# Autodesk Inventor assembly: Arm Manipulator
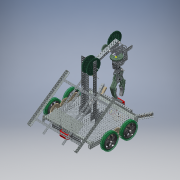
[picture p0: Inventor's stored thumbnail of the model, 180x180]
Saved by Autodesk Inventor 2018 (Build 220112000, 112)
## iProperties
Created: 2018-11-11
Part Number: Arm Manipulator
Document SubType Name: Assembly
Designer: USER
Author: USER
## Documents named in this file (32)
- C:\Users\USER\Desktop\School\Grade 12\Sem 1\Computer Engineering\Competition Robot Inventor\Vex Arm Assembly\Arm Manipulator.iam
- C:\Users\USER\Desktop\School\Grade 12\Sem 1\Computer Engineering\Competition Robot Inventor\Vex Arm Assembly\84 Tooth Gear.ipt
- C:\Users\USER\Desktop\School\Grade 12\Sem 1\Computer Engineering\Competition Robot Inventor\Vex Arm Assembly\Shaft 4 inch.ipt
- C:\Users\USER\Desktop\School\Grade 12\Sem 1\Computer Engineering\Competition Robot Inventor\Vex Arm Assembly\Shaft 3 inch.ipt
- C:\Users\USER\Desktop\School\Grade 12\Sem 1\Computer Engineering\Competition Robot Inventor\Vex Arm Assembly\36 Tooth Gear.ipt
- C:\Users\USER\Desktop\School\Grade 12\Sem 1\Computer Engineering\Competition Robot Inventor\Vex Arm Assembly\Lin Mot-Rack Brk.ipt
- C:\Users\USER\Desktop\School\Grade 12\Sem 1\Computer Engineering\Competition Robot Inventor\Vex Arm Assembly\60 Tooth Gear.ipt
- C:\Users\USER\Desktop\School\Grade 12\Sem 1\Computer Engineering\Competition Robot Inventor\Vex Arm Assembly\Pivot Gusset.ipt
- C:\Users\USER\Desktop\School\Grade 12\Sem 1\Computer Engineering\Competition Robot Inventor\Vex Arm Assembly\Hinge.iam
- C:\Users\USER\Desktop\School\Grade 12\Sem 1\Computer Engineering\Competition Robot Inventor\Vex Arm Assembly\Shaft Collar.iam
- C:\Users\USER\Desktop\School\Grade 12\Sem 1\Computer Engineering\Competition Robot Inventor\Vex Arm Assembly\Screw 8-32  x 0.375 inch long.ipt
- C:\Users\USER\Desktop\School\Grade 12\Sem 1\Computer Engineering\Competition Robot Inventor\Vex Arm Assembly\VEX Claw Finger.iam
- C:\Users\USER\Desktop\School\Grade 12\Sem 1\Computer Engineering\Competition Robot Inventor\Vex Arm Assembly\Gripper_Assembly_SubAssembly.iam
- C:\Users\USER\Desktop\School\Grade 12\Sem 1\Computer Engineering\Competition Robot Inventor\Vex Arm Assembly\VEX-12-TOOTH-GEAR.ipt
- C:\Users\USER\Desktop\School\Grade 12\Sem 1\Computer Engineering\Competition Robot Inventor\Vex Arm Assembly\Vexplorer-CLAW-GEAR-LINKAGE.ipt
- C:\Users\USER\Desktop\School\Grade 12\Sem 1\Computer Engineering\Competition Robot Inventor\Vex Arm Assembly\Vexplorer-CLAW-LINKAGE.ipt
- C:\Users\USER\Desktop\School\Grade 12\Sem 1\Computer Engineering\Competition Robot Inventor\Vex Arm Assembly\SHAFT-2000.ipt
- C:\Users\USER\Desktop\School\Grade 12\Sem 1\Computer Engineering\Competition Robot Inventor\Vex Arm Assembly\Chassis Bumper 25 Hole.ipt
- C:\Users\USER\Desktop\School\Grade 12\Sem 1\Computer Engineering\Competition Robot Inventor\Vex Arm Assembly\Plate 5x25 Hole.ipt
- C:\Users\USER\Downloads\Inventor_2013_VEX_ KOP_-_Metric\Metric\Structure\C-Channel 1x2x1x15 Hole.ipt
- C:\Users\USER\Downloads\Inventor_2013_VEX_ KOP_-_Metric\Metric\Structure\Chassis Rail 25 Hole.ipt
- C:\Users\USER\Downloads\Inventor_2013_VEX_ KOP_-_Metric\Metric\Structure\Bar 1x20.ipt
- C:\Users\USER\Downloads\Inventor_2013_VEX_ KOP_-_Metric\Metric\Motion\Bearing Flat.ipt
- C:\Users\USER\Downloads\Inventor_2013_VEX_ KOP_-_Metric\Metric\Structure\Chassis Rail 16 Hole.ipt
- C:\Users\USER\Downloads\Inventor_2013_VEX_ KOP_-_Metric\Metric\Motion\4 inch Wheel.iam
- C:\Users\USER\Downloads\Inventor_2013_VEX_ KOP_-_Metric\Metric\Motion\19 Tooth Rack Gear.ipt
- C:\Users\USER\Downloads\Inventor_2013_VEX_ KOP_-_Metric\Metric\Structure\Bar 1x25.ipt
- C:\Users\USER\Desktop\School\Grade 12\Sem 1\Computer Engineering\Competition Robot Inventor\Vex Arm Assembly\C-Channel 1x2x1x25 Hole.ipt
- C:\Users\USER\Downloads\Inventor_2013_VEX_ KOP_-_Metric\Metric\Motion\12 Tooth Gear.ipt
- C:\Users\USER\Downloads\Inventor_2013_VEX_ KOP_-_Metric\Metric\Structure\Plate 5x15 Hole.ipt
- C:\Users\USER\Downloads\Inventor_2013_VEX_ KOP_-_Metric\Metric\Sensors\Line Tracker.iam
- C:\Users\USER\Downloads\Inventor_2013_VEX_ KOP_-_Metric\Metric\Sensors\Ultrasonic Range Finder (Sensor).iam
## Components (118 placed, 31 different names)
1. 84 Tooth Gear:1 — Rigid:3, Rigid:11, Rigid:25, Rigid:26, Rotation:4
2. 84 Tooth Gear:2 — Rigid:6
3. 84 Tooth Gear:3 — Rigid:7, Rotation:10
4. Shaft 4 inch:1 — Rigid:3, Rigid:18, Rigid:19, Rotational:42
5. Shaft 4 inch:2 — Rigid:6, Rigid:7, Rigid:21, Rigid:22, Rotational:41, Rigid:42
6. Shaft 3 inch:1 — Rigid:5, Rigid:20, Rigid:31, Rotational:43
7. 36 Tooth Gear:1 — Rigid:5, Flush:1, Rotation:4
8. Lin Mot-Rack Brk:1 — Rotational:4, Rigid:11, Rigid:14
9. Lin Mot-Rack Brk:2 — Rigid:10, Rigid:15, Rigid:29, Rigid:30, Rigid:34
10. 60 Tooth Gear:1 — Rigid:9
11. Shaft 3 inch:2 — Rotational:4, Rigid:9, Rigid:10, Rotational:5, Rigid:23, Rigid:24
12. Pivot Gusset:1 — Rigid:15, Rigid:16
13. Pivot Gusset:2 — Rigid:14
14. Hinge:1 [sub-assembly] — Rigid:17
15. Hinge:2 [sub-assembly] — Rigid:16, Rigid:17
16. Shaft Collar:1 [sub-assembly] — Rigid:19
17. Shaft Collar:2 [sub-assembly] — Rigid:20
18. Shaft Collar:3 [sub-assembly] — Rigid:18
19. Shaft Collar:5 [sub-assembly] — Rigid:21
20. Shaft Collar:6 [sub-assembly] — Rotational:5
21. Shaft Collar:7 [sub-assembly] — Rigid:24
22. Shaft Collar:9 [sub-assembly] — Rigid:23
23. Shaft Collar:10 [sub-assembly] — Rigid:22
24. Hexagon Socket Button Head Cap Screw - Inch 8 - 32 x 3/8:1 — Rigid:26
25. Hexagon Socket Button Head Cap Screw - Inch 8 - 32 x 3/8:3 — Rigid:25
26. Hexagon Socket Button Head Cap Screw - Inch 8 - 32 x 3/8:5 — Rigid:29
27. Hexagon Socket Button Head Cap Screw - Inch 8 - 32 x 3/8:6 — Rigid:30
28. Shaft Collar:11 [sub-assembly] — Rigid:31
29. VEX Claw Finger:1 [sub-assembly] — Rotational:39, Rotational:40
30. VEX Claw Finger:2 [sub-assembly] — Rotational:35, Rotational:36
31. Gripper_Assembly_SubAssembly:1 [sub-assembly] — Rotational:34, Rotational:6, Rotational:7, Rotational:37, Rotational:38, Rigid:34
32. VEX-12-TOOTH-GEAR:1 — Rigid:32, Rotation:2
33. Vexplorer-CLAW-GEAR-LINKAGE:1 — Rotational:37, Rotational:39, Rotation:3
34. Vexplorer-CLAW-LINKAGE:1 — Rotational:38, Rotational:40
35. Vexplorer-CLAW-LINKAGE:2 — Rotational:7, Rotational:36
36. Vexplorer-CLAW-GEAR-LINKAGE:2 — Rotational:6, Rotation:2, Rotational:35, Rotation:3
37. SHAFT-2000:1 — Rigid:32, Rotational:34, Rigid:33
38. Shaft Collar:12 [sub-assembly] — Rigid:33
39. Chassis Bumper 25 Hole:1 — Rigid:41
40. Chassis Bumper 25 Hole:2 — Rotational:41, Rigid:39, Rotational:87
41. Plate 5x25 Hole:1 — Mate:5, Rigid:43, Rigid:50
42. Lin Mot-Rack Brk:3 — Rigid:39, Rigid:43, Rigid:49
43. Lin Mot-Rack Brk:4 — Rigid:41
44. C-Channel 1x2x1x15 Hole:1 — Rotational:42, Rotational:43, Rigid:42
45. Plate 5x25 Hole:2 — Rigid:48, Rigid:53, Rigid:54, Rotational:50, Rotational:86
46. Plate 5x25 Hole:3 — Rigid:49
47. Plate 5x25 Hole:4 — Rigid:51
48. Chassis Rail 25 Hole:1 — Rigid:45, Rigid:46
49. Chassis Rail 25 Hole:2 — Rigid:45, Rigid:48, Rigid:50, Rigid:51, Rigid:52
50. Chassis Rail 25 Hole:3 — Rigid:46, Rigid:47
51. Chassis Rail 25 Hole:4 — Rigid:47, Rigid:89, Rigid:90, Rigid:91
52. Bar 1x20:1 — Rigid:52, Rigid:92
53. Bearing Flat:1 — Rigid:55, Rotational:46
54. Bearing Flat:2 — Rigid:57, Rotational:44
55. Bearing Flat:3 — Rigid:56, Rotational:45
56. Chassis Rail 16 Hole:1 — Rigid:53, Rigid:55, Rigid:56, Rigid:57
57. Chassis Rail 16 Hole:2 — Rigid:54, Rigid:66, Rigid:67, Rigid:68
58. Shaft 4 inch:3 — Rotational:44, Rigid:58, Rigid:61, Rigid:65
59. Shaft 4 inch:4 — Rotational:45, Rigid:60, Rigid:64
60. Shaft 4 inch:5 — Rotational:46, Rigid:59, Rigid:62, Rigid:63
61. 4 inch Wheel:1 [sub-assembly] — Rigid:61
62. Shaft Collar:13 [sub-assembly] — Rigid:58
63. Shaft Collar:14 [sub-assembly] — Rigid:60
64. Shaft Collar:15 [sub-assembly] — Rigid:59
65. 4 inch Wheel:2 [sub-assembly] — Rigid:62
66. 60 Tooth Gear:2 — Rigid:63, Rotation:6
67. 60 Tooth Gear:3 — Rigid:64, Rotation:5, Rotation:6
68. 60 Tooth Gear:4 — Rigid:65, Rotation:5
69. Bearing Flat:4 — Rigid:66, Rotational:47
70. Bearing Flat:5 — Rigid:67, Rotational:48
71. Bearing Flat:6 — Rigid:68, Rotational:49
72. Shaft 4 inch:6 — Rotational:47, Rigid:69, Rigid:72, Rigid:74
73. Shaft 4 inch:7 — Rotational:48, Rigid:70, Rigid:75
74. Shaft 4 inch:8 — Rotational:49, Rigid:71, Rigid:73, Rigid:76
75. Shaft Collar:16 [sub-assembly] — Rigid:69
76. Shaft Collar:17 [sub-assembly] — Rigid:70
77. Shaft Collar:18 [sub-assembly] — Rigid:71
78. 4 inch Wheel:3 [sub-assembly] — Rigid:73
79. 4 inch Wheel:4 [sub-assembly] — Rigid:72
80. 60 Tooth Gear:5 — Rigid:74, Rotation:8
81. 60 Tooth Gear:6 — Rigid:75, Rotation:7, Rotation:8
82. 60 Tooth Gear:7 — Rigid:76, Rotation:7
83. C-Channel 1x2x1x15 Hole:2 — Rigid:77, Rigid:79, Rigid:87
84. C-Channel 1x2x1x15 Hole:3 — Rigid:78, Rigid:80, Rigid:88
85. 60 Tooth Gear:8 — Rigid:77, Rotation:9
86. 60 Tooth Gear:9 — Rigid:78, Rotation:9
87. Bearing Flat:7 — Rigid:79, Rigid:81
88. Bearing Flat:8 — Rigid:80, Rigid:82
89. Shaft 3 inch:3 — Rigid:82, Rigid:84, Rotational:86, Rigid:85
90. Shaft 3 inch:4 — Rigid:81, Rigid:83, Rotational:50, Rigid:86
91. Shaft Collar:19 [sub-assembly] — Rigid:83
92. Shaft Collar:20 [sub-assembly] — Rigid:84
93. Shaft Collar:21 [sub-assembly] — Rigid:85
94. Shaft Collar:22 [sub-assembly] — Rigid:86
95. 19 Tooth Rack Gear:1 — Rigid:87
96. 19 Tooth Rack Gear:2 — Rigid:88
97. Bar 1x25:1 — Rigid:90
98. Bar 1x25:2 — Rigid:89, Rigid:104
99. C-Channel 1x2x1x15 Hole:4 — Rigid:91, Rigid:110
100. C-Channel 1x2x1x25 Hole:1 — Rigid:92, Rigid:109
101. 12 Tooth Gear:1 — Rigid:93
102. 12 Tooth Gear:2 — Rigid:94, Rotation:10
103. Shaft 4 inch:9 — Rotational:87, Rigid:93, Rigid:94, Rigid:95, Rigid:96
104. Shaft Collar:23 [sub-assembly] — Rigid:95
105. Shaft Collar:24 [sub-assembly] — Rigid:96
106. Chassis Rail 25 Hole:5 — Rigid:97, Rigid:99, Rigid:100
107. Chassis Rail 25 Hole:6 — Rigid:98
108. Bar 1x20:2 — Rigid:97, Rigid:98, Rigid:99, Rigid:101, Rigid:102, Rigid:104
109. Bar 1x20:3 — Rigid:101, Rigid:103
110. Bar 1x20:4 — Rigid:102
111. Bar 1x20:5 — Rigid:100
112. Plate 5x15 Hole:1 — Rigid:103
113. C-Channel 1x2x1x15 Hole:5 — Rigid:105, Rigid:106, Rigid:107, Rigid:108, Rigid:109
114. Line Tracker:1 [sub-assembly] — Rigid:105
115. Line Tracker:2 [sub-assembly] — Rigid:106
116. Line Tracker:3 [sub-assembly] — Rigid:107
117. Ultrasonic Range Finder (Sensor):1 [sub-assembly] — Rigid:110
118. Ultrasonic Range Finder (Sensor):2 [sub-assembly] — Rigid:108
## Relationships (130: WeldJoint 96, RevoluteJoint 23, RelateRotation 9, Flush 1, Mate 1)
- Rigid:3 [WeldJoint] (36.5125 mm): 84 Tooth Gear:1 ↔ Shaft 4 inch:1
- Rigid:5 [WeldJoint] (-16.51 mm): Shaft 3 inch:1 ↔ 36 Tooth Gear:1
- Rigid:6 [WeldJoint] (-31.75 mm): 84 Tooth Gear:2 ↔ Shaft 4 inch:2
- Rigid:7 [WeldJoint] (-25.4 mm): 84 Tooth Gear:3 ↔ Shaft 4 inch:2
- Rotational:4 [RevoluteJoint] (-10 mm): Lin Mot-Rack Brk:1 ↔ Shaft 3 inch:2
- Rigid:9 [WeldJoint] (-20 mm): 60 Tooth Gear:1 ↔ Shaft 3 inch:2
- Rigid:10 [WeldJoint] (15 mm): Lin Mot-Rack Brk:2 ↔ Shaft 3 inch:2
- Rigid:11 [WeldJoint]: 84 Tooth Gear:1 ↔ Lin Mot-Rack Brk:1
- Rigid:14 [WeldJoint]: Lin Mot-Rack Brk:1 ↔ Pivot Gusset:2
- Rigid:15 [WeldJoint]: Lin Mot-Rack Brk:2 ↔ Pivot Gusset:1
- Rigid:16 [WeldJoint]: Pivot Gusset:1 ↔ Hinge:2
- Rigid:17 [WeldJoint]: Hinge:1 ↔ Hinge:2
- Rigid:18 [WeldJoint] (-12.7 mm): Shaft 4 inch:1 ↔ Shaft Collar:3
- Rigid:19 [WeldJoint] (-38.1 mm): Shaft 4 inch:1 ↔ Shaft Collar:1
- Rigid:20 [WeldJoint] (-6.35 mm): Shaft 3 inch:1 ↔ Shaft Collar:2
- Rigid:21 [WeldJoint] (-25.4 mm): Shaft 4 inch:2 ↔ Shaft Collar:5
- Rigid:22 [WeldJoint] (-25.4 mm): Shaft 4 inch:2 ↔ Shaft Collar:10
- Rotational:5 [RevoluteJoint] (-3.175 mm): Shaft 3 inch:2 ↔ Shaft Collar:6
- Rigid:23 [WeldJoint] (-9.525 mm): Shaft 3 inch:2 ↔ Shaft Collar:9
- Rigid:24 [WeldJoint] (-14.2875 mm): Shaft 3 inch:2 ↔ Shaft Collar:7
- Rigid:25 [WeldJoint] (-7.9375 mm): 84 Tooth Gear:1 ↔ Hexagon Socket Button Head Cap Screw - Inch 8 - 32 x 3/8:3
- Rigid:26 [WeldJoint] (-9.525 mm): 84 Tooth Gear:1 ↔ Hexagon Socket Button Head Cap Screw - Inch 8 - 32 x 3/8:1
- Rigid:29 [WeldJoint] (-7.9375 mm): Lin Mot-Rack Brk:2 ↔ Hexagon Socket Button Head Cap Screw - Inch 8 - 32 x 3/8:5
- Rigid:30 [WeldJoint] (-7.9375 mm): Lin Mot-Rack Brk:2 ↔ Hexagon Socket Button Head Cap Screw - Inch 8 - 32 x 3/8:6
- Rigid:31 [WeldJoint] (1.5875 mm): Shaft 3 inch:1 ↔ Shaft Collar:11
- Rigid:32 [WeldJoint] (-20.6375 mm): VEX-12-TOOTH-GEAR:1 ↔ SHAFT-2000:1
- Rotational:34 [RevoluteJoint] (31.75 mm): Gripper_Assembly_SubAssembly:1 ↔ SHAFT-2000:1
- Rotational:6 [RevoluteJoint]: Gripper_Assembly_SubAssembly:1 ↔ Vexplorer-CLAW-GEAR-LINKAGE:2
- Rotation:2 [RelateRotation] (1 ul): VEX-12-TOOTH-GEAR:1 ↔ Vexplorer-CLAW-GEAR-LINKAGE:2
- Rotational:7 [RevoluteJoint]: Gripper_Assembly_SubAssembly:1 ↔ Vexplorer-CLAW-LINKAGE:2
- Rotational:35 [RevoluteJoint]: VEX Claw Finger:2 ↔ Vexplorer-CLAW-GEAR-LINKAGE:2
- Rotational:36 [RevoluteJoint]: VEX Claw Finger:2 ↔ Vexplorer-CLAW-LINKAGE:2
- Rotational:37 [RevoluteJoint]: Gripper_Assembly_SubAssembly:1 ↔ Vexplorer-CLAW-GEAR-LINKAGE:1
- Rotational:38 [RevoluteJoint]: Gripper_Assembly_SubAssembly:1 ↔ Vexplorer-CLAW-LINKAGE:1
- Rotational:39 [RevoluteJoint]: VEX Claw Finger:1 ↔ Vexplorer-CLAW-GEAR-LINKAGE:1
- Rotational:40 [RevoluteJoint]: VEX Claw Finger:1 ↔ Vexplorer-CLAW-LINKAGE:1
- Rigid:33 [WeldJoint] (-17.4625 mm): SHAFT-2000:1 ↔ Shaft Collar:12
- Rigid:34 [WeldJoint]: Lin Mot-Rack Brk:2 ↔ Gripper_Assembly_SubAssembly:1
- Rotation:3 [RelateRotation] (1 ul): Vexplorer-CLAW-GEAR-LINKAGE:1 ↔ Vexplorer-CLAW-GEAR-LINKAGE:2
- Rotational:41 [RevoluteJoint] (25.4 mm): Shaft 4 inch:2 ↔ Chassis Bumper 25 Hole:2
- Rigid:39 [WeldJoint]: Chassis Bumper 25 Hole:2 ↔ Lin Mot-Rack Brk:3
- Rigid:41 [WeldJoint]: Chassis Bumper 25 Hole:1 ↔ Lin Mot-Rack Brk:4
- Flush:1 (-3.81 mm): 36 Tooth Gear:1
- Mate:5: Plate 5x25 Hole:1
- Rotational:42 [RevoluteJoint] (-39.6875 mm): Shaft 4 inch:1 ↔ C-Channel 1x2x1x15 Hole:1
- Rotational:43 [RevoluteJoint] (15.875 mm): Shaft 3 inch:1 ↔ C-Channel 1x2x1x15 Hole:1
- Rigid:42 [WeldJoint] (-38.1 mm): Shaft 4 inch:2 ↔ C-Channel 1x2x1x15 Hole:1
- Rotation:4 [RelateRotation] (1 ul): 84 Tooth Gear:1 ↔ 36 Tooth Gear:1
- Rigid:43 [WeldJoint]: Plate 5x25 Hole:1 ↔ Lin Mot-Rack Brk:3
- Rigid:45 [WeldJoint]: Chassis Rail 25 Hole:1 ↔ Chassis Rail 25 Hole:2
- Rigid:46 [WeldJoint]: Chassis Rail 25 Hole:1 ↔ Chassis Rail 25 Hole:3
- Rigid:47 [WeldJoint]: Chassis Rail 25 Hole:3 ↔ Chassis Rail 25 Hole:4
- Rigid:48 [WeldJoint]: Plate 5x25 Hole:2 ↔ Chassis Rail 25 Hole:2
- Rigid:49 [WeldJoint]: Lin Mot-Rack Brk:3 ↔ Plate 5x25 Hole:3
- Rigid:50 [WeldJoint]: Plate 5x25 Hole:1 ↔ Chassis Rail 25 Hole:2
- Rigid:51 [WeldJoint]: Plate 5x25 Hole:4 ↔ Chassis Rail 25 Hole:2
- Rigid:52 [WeldJoint]: Chassis Rail 25 Hole:2 ↔ Bar 1x20:1
- Rigid:53 [WeldJoint]: Plate 5x25 Hole:2 ↔ Chassis Rail 16 Hole:1
- Rigid:54 [WeldJoint]: Plate 5x25 Hole:2 ↔ Chassis Rail 16 Hole:2
- Rigid:55 [WeldJoint]: Bearing Flat:1 ↔ Chassis Rail 16 Hole:1
- Rigid:56 [WeldJoint]: Bearing Flat:3 ↔ Chassis Rail 16 Hole:1
- Rigid:57 [WeldJoint]: Bearing Flat:2 ↔ Chassis Rail 16 Hole:1
- Rotational:44 [RevoluteJoint] (-23.8125 mm): Bearing Flat:2 ↔ Shaft 4 inch:3
- Rotational:45 [RevoluteJoint] (-23.8125 mm): Bearing Flat:3 ↔ Shaft 4 inch:4
- Rotational:46 [RevoluteJoint] (-23.8125 mm): Bearing Flat:1 ↔ Shaft 4 inch:5
- Rigid:58 [WeldJoint] (-7.9375 mm): Shaft 4 inch:3 ↔ Shaft Collar:13
- Rigid:60 [WeldJoint] (-30.1625 mm): Shaft 4 inch:4 ↔ Shaft Collar:14
- Rigid:59 [WeldJoint] (-7.9375 mm): Shaft 4 inch:5 ↔ Shaft Collar:15
- Rigid:61 [WeldJoint] (-7.9375 mm): Shaft 4 inch:3 ↔ 4 inch Wheel:1
- Rigid:62 [WeldJoint] (-7.9375 mm): Shaft 4 inch:5 ↔ 4 inch Wheel:2
- Rigid:63 [WeldJoint] (-30.1625 mm): Shaft 4 inch:5 ↔ 60 Tooth Gear:2
- Rigid:64 [WeldJoint] (-30.1625 mm): Shaft 4 inch:4 ↔ 60 Tooth Gear:3
- Rigid:65 [WeldJoint] (-30.1625 mm): Shaft 4 inch:3 ↔ 60 Tooth Gear:4
- Rotation:5 [RelateRotation] (1 ul): 60 Tooth Gear:3 ↔ 60 Tooth Gear:4
- Rotation:6 [RelateRotation] (1 ul): 60 Tooth Gear:2 ↔ 60 Tooth Gear:3
- Rigid:66 [WeldJoint]: Chassis Rail 16 Hole:2 ↔ Bearing Flat:4
- Rigid:67 [WeldJoint]: Chassis Rail 16 Hole:2 ↔ Bearing Flat:5
- Rigid:68 [WeldJoint]: Chassis Rail 16 Hole:2 ↔ Bearing Flat:6
- Rotational:47 [RevoluteJoint] (23.8125 mm): Bearing Flat:4 ↔ Shaft 4 inch:6
- Rotational:48 [RevoluteJoint] (-23.8125 mm): Bearing Flat:5 ↔ Shaft 4 inch:7
- Rotational:49 [RevoluteJoint] (-23.8125 mm): Bearing Flat:6 ↔ Shaft 4 inch:8
- Rigid:69 [WeldJoint] (-7.9375 mm): Shaft 4 inch:6 ↔ Shaft Collar:16
- Rigid:70 [WeldJoint] (-28.575 mm): Shaft 4 inch:7 ↔ Shaft Collar:17
- Rigid:71 [WeldJoint] (-7.9375 mm): Shaft 4 inch:8 ↔ Shaft Collar:18
- Rigid:72 [WeldJoint] (25.4 mm): Shaft 4 inch:6 ↔ 4 inch Wheel:4
- Rigid:73 [WeldJoint] (-25.4 mm): Shaft 4 inch:8 ↔ 4 inch Wheel:3
- Rigid:74 [WeldJoint] (38.1 mm): Shaft 4 inch:6 ↔ 60 Tooth Gear:5
- Rigid:75 [WeldJoint] (-38.1 mm): Shaft 4 inch:7 ↔ 60 Tooth Gear:6
- Rigid:76 [WeldJoint] (38.1 mm): Shaft 4 inch:8 ↔ 60 Tooth Gear:7
- Rotation:7 [RelateRotation] (1 ul): 60 Tooth Gear:6 ↔ 60 Tooth Gear:7
- Rotation:8 [RelateRotation] (1 ul): 60 Tooth Gear:5 ↔ 60 Tooth Gear:6
- Rigid:77 [WeldJoint]: C-Channel 1x2x1x15 Hole:2 ↔ 60 Tooth Gear:8
- Rigid:78 [WeldJoint]: C-Channel 1x2x1x15 Hole:3 ↔ 60 Tooth Gear:9
- Rigid:79 [WeldJoint]: C-Channel 1x2x1x15 Hole:2 ↔ Bearing Flat:7
- Rigid:80 [WeldJoint]: C-Channel 1x2x1x15 Hole:3 ↔ Bearing Flat:8
- Rigid:81 [WeldJoint] (42.8625 mm): Bearing Flat:7 ↔ Shaft 3 inch:4
- Rigid:82 [WeldJoint] (-9.525 mm): Bearing Flat:8 ↔ Shaft 3 inch:3
- Rigid:83 [WeldJoint] (-7.9375 mm): Shaft 3 inch:4 ↔ Shaft Collar:19
- Rigid:84 [WeldJoint] (-9.525 mm): Shaft 3 inch:3 ↔ Shaft Collar:20
- Rotational:50 [RevoluteJoint] (22.225 mm): Plate 5x25 Hole:2 ↔ Shaft 3 inch:4
- Rotational:86 [RevoluteJoint] (22.225 mm): Plate 5x25 Hole:2 ↔ Shaft 3 inch:3
- Rotation:9 [RelateRotation] (1 ul): 60 Tooth Gear:8 ↔ 60 Tooth Gear:9
- Rigid:85 [WeldJoint] (-22.225 mm): Shaft 3 inch:3 ↔ Shaft Collar:21
- Rigid:86 [WeldJoint] (-22.225 mm): Shaft 3 inch:4 ↔ Shaft Collar:22
- Rigid:87 [WeldJoint]: C-Channel 1x2x1x15 Hole:2 ↔ 19 Tooth Rack Gear:1
- Rigid:88 [WeldJoint]: C-Channel 1x2x1x15 Hole:3 ↔ 19 Tooth Rack Gear:2
- Rigid:89 [WeldJoint]: Chassis Rail 25 Hole:4 ↔ Bar 1x25:2
- Rigid:90 [WeldJoint]: Chassis Rail 25 Hole:4 ↔ Bar 1x25:1
- Rigid:91 [WeldJoint]: Chassis Rail 25 Hole:4 ↔ C-Channel 1x2x1x15 Hole:4
- Rigid:92 [WeldJoint]: Bar 1x20:1 ↔ C-Channel 1x2x1x25 Hole:1
- Rotational:87 [RevoluteJoint] (23.8125 mm): Chassis Bumper 25 Hole:2 ↔ Shaft 4 inch:9
- Rigid:93 [WeldJoint] (-61.9125 mm): 12 Tooth Gear:1 ↔ Shaft 4 inch:9
- Rigid:94 [WeldJoint] (-30.1625 mm): 12 Tooth Gear:2 ↔ Shaft 4 inch:9
- Rotation:10 [RelateRotation] (1 ul): 84 Tooth Gear:3 ↔ 12 Tooth Gear:2
- Rigid:95 [WeldJoint] (-17.4625 mm): Shaft 4 inch:9 ↔ Shaft Collar:23
- Rigid:96 [WeldJoint] (25.4 mm): Shaft 4 inch:9 ↔ Shaft Collar:24
- Rigid:97 [WeldJoint]: Chassis Rail 25 Hole:5 ↔ Bar 1x20:2
- Rigid:98 [WeldJoint]: Chassis Rail 25 Hole:6 ↔ Bar 1x20:2
- Rigid:99 [WeldJoint]: Chassis Rail 25 Hole:5 ↔ Bar 1x20:2
- Rigid:100 [WeldJoint]: Chassis Rail 25 Hole:5 ↔ Bar 1x20:5
- Rigid:101 [WeldJoint]: Bar 1x20:2 ↔ Bar 1x20:3
- Rigid:102 [WeldJoint]: Bar 1x20:2 ↔ Bar 1x20:4
- Rigid:103 [WeldJoint]: Bar 1x20:3 ↔ Plate 5x15 Hole:1
- Rigid:104 [WeldJoint]: Bar 1x25:2 ↔ Bar 1x20:2
- Rigid:105 [WeldJoint]: C-Channel 1x2x1x15 Hole:5 ↔ Line Tracker:1
- Rigid:106 [WeldJoint]: C-Channel 1x2x1x15 Hole:5 ↔ Line Tracker:2
- Rigid:107 [WeldJoint]: C-Channel 1x2x1x15 Hole:5 ↔ Line Tracker:3
- Rigid:108 [WeldJoint]: C-Channel 1x2x1x15 Hole:5 ↔ Ultrasonic Range Finder (Sensor):2
- Rigid:109 [WeldJoint]: C-Channel 1x2x1x25 Hole:1 ↔ C-Channel 1x2x1x15 Hole:5
- Rigid:110 [WeldJoint]: C-Channel 1x2x1x15 Hole:4 ↔ Ultrasonic Range Finder (Sensor):1
